# Autodesk Inventor assembly: Chest Assembly
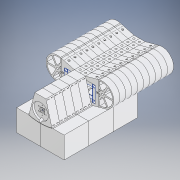
[picture p0: Inventor's stored thumbnail of the model, 180x180]
Saved by Autodesk Inventor 2017 SP1 (Build 210196100, 196)
## iProperties
Created: 2017-06-04
Part Number: Chest Assembly
Document SubType Name: Assembly
Designer: Zach
Author: Zach
## Documents named in this file (5)
- C:\Users\Zach\Documents\GitHub\tr1\src\Body\Chest Assembly\Chest Assembly.iam
- C:\Users\Zach\Documents\GitHub\tr1\src\Body\Chest Assembly\Rise Base Assembly\Riser Base.iam
- C:\Users\Zach\Documents\GitHub\tr1\src\Body\Chest Assembly\Chassis\Chassis.iam
- C:\Users\Zach\Documents\GitHub\tr1\src\Body\Chest Assembly\Backpack Assembly\Backpack.iam
- C:\Users\Zach\Documents\GitHub\tr1\src\Body\Chest Assembly\Sternum Assembly\Sternum Assembly.iam
## Components (4 placed, 4 different names)
1. Riser Base:1 [sub-assembly] — Mate:16, Mate:17, Mate:18, Mate:19, Mate:20
2. Chassis:1 [sub-assembly] — Mate:16, Mate:17
3. Backpack:1 [sub-assembly] — Mate:21, Mate:22, Mate:23
4. Sternum Assembly:1 [sub-assembly] — Mate:18, Mate:19, Mate:20, Mate:21, Mate:22, Mate:23
## Relationships (8: Mate 8)
- Mate:16: Riser Base:1 ↔ Chassis:1
- Mate:17: Riser Base:1 ↔ Chassis:1
- Mate:18: Riser Base:1 ↔ Sternum Assembly:1
- Mate:19: Riser Base:1 ↔ Sternum Assembly:1
- Mate:20: Riser Base:1 ↔ Sternum Assembly:1
- Mate:21: Backpack:1 ↔ Sternum Assembly:1
- Mate:22: Backpack:1 ↔ Sternum Assembly:1
- Mate:23: Backpack:1 ↔ Sternum Assembly:1
